# Autodesk Inventor assembly: Интерьер
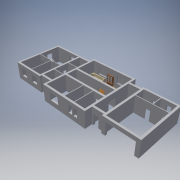
[picture p0: Inventor's stored thumbnail of the model, 180x180]
Saved by Autodesk Inventor 2019 (Build 230136000, 136)
## iProperties
Created: 2018-09-22
Part Number: Интерьер
Material: Типовые
Document SubType Name: Assembly
Designer: Андреев Н.Л.
Mass: 2.90538e+08 g
Surface Area: 1.29529e+07 cm^2
Volume: 1.64308e+08 cm^3
Density: 1.76825 g/cm^3
Author: Андреев Н.Л.
## Documents named in this file (12)
- C:\Users\andrnl\Documents\Inventor\Мурзин\Интерьер.iam
- C:\Users\andrnl\Documents\Inventor\Мурзин\Этаж 1.iam
- C:\Users\andrnl\Documents\Inventor\Мурзин\Шкаф 1дв.iam
- C:\Users\andrnl\Documents\Inventor\Мурзин\Тумба ТВ.iam
- C:\Users\andrnl\Documents\Inventor\Мурзин\Диван угловой.ipt
- C:\Users\andrnl\Documents\Inventor\Мурзин\Столик круглый.ipt
- C:\Users\andrnl\Documents\Inventor\ШР Мебель 2016\Зал\Столик теле.iam
- C:\Users\andrnl\Documents\Inventor\Мурзин\Камин.ipt
- C:\Users\andrnl\Documents\Inventor\Мурзин\Кресло простое.iam
- C:\Users\andrnl\Documents\Inventor\ШР Мебель 2016\Кабинет\Шкаф двухстворчатый СБ.iam
- C:\Users\andrnl\Documents\Inventor\ШР Мебель 2016\Кухня\Столик сервировочный.iam
- C:\Users\andrnl\Documents\Inventor\Мурзин\Бра.ipt
## Components (14 placed, 11 different names)
1. Этаж 1:1 [sub-assembly] — Заподлицо:1, Совмещение:1, Совмещение:2, Заподлицо:2, Совмещение:3, Заподлицо:3, Совмещение:5, Заподлицо:4, Совмещение:7, Совмещение:8, Заподлицо:5, Заподлицо:6, Заподлицо:7, Совмещение:9, Заподлицо:8, Заподлицо:9, Заподлицо:11, Совмещение:10, Заподлицо:12, Совмещение:11, Заподлицо:13, Совмещение:13, Заподлицо:15
2. Шкаф 1дв:1 [sub-assembly] — Заподлицо:1, Совмещение:1, Совмещение:2, Совмещение:4
3. Шкаф 1дв:2 [sub-assembly] — Заподлицо:2, Совмещение:3, Совмещение:4, Совмещение:6
4. Тумба ТВ:1 [sub-assembly] — Заподлицо:3, Совмещение:5, Совмещение:6
5. Диван угловой:1 — Заподлицо:4, Совмещение:7, Совмещение:8
6. Столик круглый:1 — Заподлицо:5
7. Столик теле:1 [sub-assembly] — Заподлицо:6
8. Камин:1 — Заподлицо:7, Совмещение:9, Совмещение:12, Заподлицо:14
9. Кресло простое:1 [sub-assembly] — Заподлицо:8
10. Кресло простое:2 [sub-assembly] — Заподлицо:9
11. Шкаф двухстворчатый СБ:1 [sub-assembly] — Заподлицо:11, Совмещение:10
12. Столик сервировочный:1 [sub-assembly] — Заподлицо:12
13. Бра:1 — Совмещение:11, Совмещение:12, Заподлицо:13
14. Бра:2 — Совмещение:13, Заподлицо:14, Заподлицо:15
## Relationships (27: Flush 14, Mate 13)
- Заподлицо:1 [Flush]: Этаж 1:1 ↔ Шкаф 1дв:1
- Совмещение:1 [Mate]: Этаж 1:1 ↔ Шкаф 1дв:1
- Совмещение:2 [Mate] (650 mm): Этаж 1:1 ↔ Шкаф 1дв:1
- Заподлицо:2 [Flush]: Этаж 1:1 ↔ Шкаф 1дв:2
- Совмещение:3 [Mate]: Этаж 1:1 ↔ Шкаф 1дв:2
- Совмещение:4 [Mate] (1700 mm): Шкаф 1дв:1 ↔ Шкаф 1дв:2
- Заподлицо:3 [Flush]: Этаж 1:1 ↔ Тумба ТВ:1
- Совмещение:5 [Mate]: Этаж 1:1 ↔ Тумба ТВ:1
- Совмещение:6 [Mate] (100 mm): Шкаф 1дв:2 ↔ Тумба ТВ:1
- Заподлицо:4 [Flush]: Этаж 1:1 ↔ Диван угловой:1
- Совмещение:7 [Mate] (100 mm): Этаж 1:1 ↔ Диван угловой:1
- Совмещение:8 [Mate] (200 mm): Этаж 1:1 ↔ Диван угловой:1
- Заподлицо:5 [Flush]: Этаж 1:1 ↔ Столик круглый:1
- Заподлицо:6 [Flush]: Этаж 1:1 ↔ Столик теле:1
- Заподлицо:7 [Flush]: Этаж 1:1 ↔ Камин:1
- Совмещение:9 [Mate]: Этаж 1:1 ↔ Камин:1
- Заподлицо:8 [Flush]: Этаж 1:1 ↔ Кресло простое:1
- Заподлицо:9 [Flush]: Этаж 1:1 ↔ Кресло простое:2
- Заподлицо:11 [Flush]: Этаж 1:1 ↔ Шкаф двухстворчатый СБ:1
- Совмещение:10 [Mate] (250 mm): Этаж 1:1 ↔ Шкаф двухстворчатый СБ:1
- Заподлицо:12 [Flush]: Этаж 1:1 ↔ Столик сервировочный:1
- Совмещение:11 [Mate]: Этаж 1:1 ↔ Бра:1
- Совмещение:12 [Mate] (500 mm): Камин:1 ↔ Бра:1
- Заподлицо:13 [Flush] (-1800 mm): Этаж 1:1 ↔ Бра:1
- Совмещение:13 [Mate]: Этаж 1:1 ↔ Бра:2
- Заподлицо:14 [Flush] (-500 mm): Камин:1 ↔ Бра:2
- Заподлицо:15 [Flush] (-1800 mm): Этаж 1:1 ↔ Бра:2
